# Autodesk Inventor assembly: case_assembly2
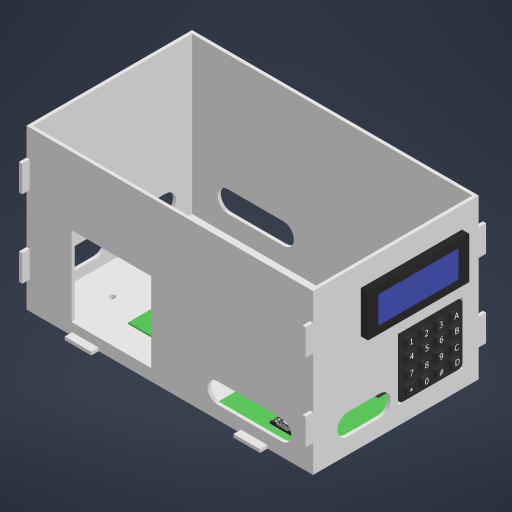
[picture p0: Inventor's stored thumbnail of the model, 512x512]
Saved by Autodesk Inventor 2023 (Build 270158000, 158)
## iProperties
Created: 2022-11-27
Part Number: case_assembly2
Document SubType Name: Assembly
Designer: washington
Author: washington
## Documents named in this file (10)
- C:\Users\washi\Desktop\FYP18-22\ELECTRONICS_CAD\case_assembly2.iam
- C:\Users\washi\Desktop\FYP18-22\ELECTRONICS_CAD\lcd\LCD_I2C\Lcd i2c.iam
- C:\Users\washi\Desktop\FYP18-22\ELECTRONICS_CAD\perspex_shell_to_cut\front_part.ipt
- C:\Users\washi\Desktop\FYP18-22\ELECTRONICS_CAD\keypad\keypad 4x4.ipt
- C:\Users\washi\Desktop\FYP18-22\ELECTRONICS_CAD\perspex_shell_to_cut\side_part.ipt
- C:\Users\washi\Desktop\FYP18-22\ELECTRONICS_CAD\perspex_shell_to_cut\back_part.ipt
- C:\Users\washi\Desktop\FYP18-22\ELECTRONICS_CAD\perspex_shell_to_cut\side_part2.ipt
- C:\Users\washi\Desktop\FYP18-22\ELECTRONICS_CAD\perspex_shell_to_cut\bottom_part.ipt
- C:\Users\washi\Desktop\FYP18-22\ELECTRONICS_CAD\pcbs\triac_pcb\TRIAC_SWITCHING.iam
- C:\Users\washi\Desktop\FYP18-22\ELECTRONICS_CAD\pcbs\Electronic design.iam
## Components (9 placed, 9 different names)
1. Lcd i2c:1 [sub-assembly] — Mate:1, Mate:2, Mate:3
2. front_part:1 — Mate:1, Mate:2, Mate:3, Mate:4, Mate:5, Mate:6, Mate:7, Mate:8, Mate:12, Mate:13, Mate:14, Mate:17
3. keypad 4x4:1 — Mate:4, Mate:5, Mate:17
4. side_part:1 — Mate:6, Mate:7, Mate:8, Mate:15, Mate:16, Mate:18
5. back_part:1 — Mate:15, Mate:16, Mate:20
6. side_part2:1 — Mate:12, Mate:13, Mate:14, Mate:19
7. bottom_part:1 — Mate:18, Mate:19, Mate:20, Mate:21, Mate:23, Mate:24, Mate:26, Mate:27, Mate:28
8. TRIAC_SWITCHING:1 [sub-assembly] — Mate:21, Mate:26, Mate:28
9. Electronic design:1 [sub-assembly] — Mate:23, Mate:24, Mate:27
## Relationships (23: Mate 23)
- Mate:1: Lcd i2c:1 ↔ front_part:1
- Mate:2: Lcd i2c:1 ↔ front_part:1
- Mate:3: Lcd i2c:1 ↔ front_part:1
- Mate:4: front_part:1 ↔ keypad 4x4:1
- Mate:5: front_part:1 ↔ keypad 4x4:1
- Mate:6: front_part:1 ↔ side_part:1
- Mate:7: front_part:1 ↔ side_part:1
- Mate:8: front_part:1 ↔ side_part:1
- Mate:12: front_part:1 ↔ side_part2:1
- Mate:13: front_part:1 ↔ side_part2:1
- Mate:14: front_part:1 ↔ side_part2:1
- Mate:15: side_part:1 ↔ back_part:1
- Mate:16: side_part:1 ↔ back_part:1
- Mate:17: front_part:1 ↔ keypad 4x4:1
- Mate:18: side_part:1 ↔ bottom_part:1
- Mate:19: side_part2:1 ↔ bottom_part:1
- Mate:20: back_part:1 ↔ bottom_part:1
- Mate:21: bottom_part:1 ↔ TRIAC_SWITCHING:1
- Mate:23: bottom_part:1 ↔ Electronic design:1
- Mate:24: bottom_part:1 ↔ Electronic design:1
- Mate:26: bottom_part:1 ↔ TRIAC_SWITCHING:1
- Mate:27: bottom_part:1 ↔ Electronic design:1
- Mate:28: bottom_part:1 ↔ TRIAC_SWITCHING:1
